# Autodesk Inventor assembly: ASM - CDROM
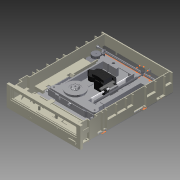
[picture p0: Inventor's stored thumbnail of the model, 180x180]
Saved by Autodesk Inventor 2011 (Build 150239000, 239)
## iProperties
Created: 2011-02-24
Part Number: ASM - CDROM
Document SubType Name: Assembly
Designer: nawrocm
Translation Standard: STEP AP214IS
FileName: C:/Users/nawrocm/Desktop/DVD Drive Finale_with_thread_removed.stp
PreProcessor: Unknown
PostProcessor: Build: 239, Release: 2011 RTM - Date: Wed 02/17/2010
Sent Units: millimeter
Uncertainty: 0.001
Author: nawrocm
## Documents named in this file (11)
- E:\3\ASM - CDROM.iam
- E:\3\MotorTray.ipt
- E:\3\Plastic Brace.ipt
- E:\3\Case Top.ipt
- E:\3\Case front.ipt
- E:\3\Case Bottom.ipt
- E:\3\Assembley.iam
- E:\3\Drive Base.iam
- E:\3\Laser.iam
- E:\3\final assembly.iam
- E:\3\rack2.ipt
## Components (10 placed, 10 different names)
1. MotorTray:1 — Flush:2, Mate:9, Mate:10, Angle:1, Mate:12, Mate:13, Flush:3, Mate:14
2. Plastic Brace:1 — Mate:5, Mate:6, Flush:2, Mate:9, Mate:12
3. Case Top:1 — Mate:20, Mate:21, Mate:22, Mate:23
4. Case front:1 — Mate:3, Mate:4, Mate:8, Mate:22, Mate:23
5. Case Bottom:1 — Mate:1, Flush:1, Mate:2, Mate:7, Mate:11, Mate:15, Mate:20, Mate:21
6. Assembley:1 [sub-assembly] — Mate:10, Angle:1, Mate:11
7. Drive Base:1 [sub-assembly] — Mate:1, Flush:1, Mate:2, Mate:3, Mate:4, Mate:5, Mate:6, Mate:7, Mate:8, Mate:16, Mate:17
8. Laser:1 [sub-assembly] — Mate:13, Flush:3, Mate:14, Flush:4, Mate:18, Mate:19
9. final assembly:1 [sub-assembly] — Mate:15, Mate:16, Mate:17
10. rack2:1 — Flush:4, Mate:18, Mate:19
## Relationships (28: Mate 23, Flush 4, Angle 1)
- Mate:1: Case Bottom:1 ↔ Drive Base:1
- Flush:1: Case Bottom:1 ↔ Drive Base:1
- Mate:2: Case Bottom:1 ↔ Drive Base:1
- Mate:3: Case front:1 ↔ Drive Base:1
- Mate:4: Case front:1 ↔ Drive Base:1
- Mate:5: Plastic Brace:1 ↔ Drive Base:1
- Mate:6: Plastic Brace:1 ↔ Drive Base:1
- Flush:2: MotorTray:1 ↔ Plastic Brace:1
- Mate:7: Case Bottom:1 ↔ Drive Base:1
- Mate:8: Case front:1 ↔ Drive Base:1
- Mate:9: MotorTray:1 ↔ Plastic Brace:1
- Mate:10: MotorTray:1 ↔ Assembley:1
- Angle:1 (0 deg): MotorTray:1 ↔ Assembley:1
- Mate:11: Case Bottom:1 ↔ Assembley:1
- Mate:12: MotorTray:1 ↔ Plastic Brace:1
- Mate:13: MotorTray:1 ↔ Laser:1
- Flush:3: MotorTray:1 ↔ Laser:1
- Mate:14: MotorTray:1 ↔ Laser:1
- Mate:15: Case Bottom:1 ↔ final assembly:1
- Mate:16: Drive Base:1 ↔ final assembly:1
- Mate:17: Drive Base:1 ↔ final assembly:1
- Flush:4: Laser:1 ↔ rack2:1
- Mate:18: Laser:1 ↔ rack2:1
- Mate:19: Laser:1 ↔ rack2:1
- Mate:20: Case Top:1 ↔ Case Bottom:1
- Mate:21: Case Top:1 ↔ Case Bottom:1
- Mate:22: Case Top:1 ↔ Case front:1
- Mate:23: Case Top:1 ↔ Case front:1
